# Autodesk Inventor assembly: タミヤダンパーフロント56,74.5
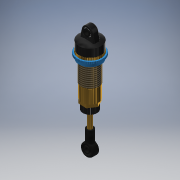
[picture p0: Inventor's stored thumbnail of the model, 180x180]
Saved by Autodesk Inventor 2020 (Build 240168000, 168)
## iProperties
Part Number: タミヤダンパーフロント56,74.5
Material: 一般
Document SubType Name: Assembly
Designer: 雪村
Mass: 29.9788 g
Surface Area: 59.981 cm^2
Volume: 5.28575 cm^3
Density: 5.67163 g/cm^3
Author: 雪村
## Documents named in this file (9)
- C:\Users\white\Documents\SRDC\SRDC\Inventor_2017\2018年機体\パーツ\タミヤダンパーフロント56,74.5.iam
- C:\Users\white\Documents\SRDC\SRDC\Inventor_2017\2018年機体\パーツ\タミヤダンパー1.ipt
- C:\Users\white\Documents\SRDC\SRDC\Inventor_2017\2018年機体\パーツ\タミヤダンパー2.ipt
- C:\Users\white\Documents\SRDC\SRDC\Inventor_2017\2018年機体\パーツ\タミヤダンパー3.ipt
- C:\Users\white\Documents\SRDC\SRDC\Inventor_2017\2018年機体\パーツ\タミヤダンパー4.ipt
- C:\Users\white\Documents\SRDC\SRDC\Inventor_2017\2018年機体\パーツ\タミヤダンパー6.ipt
- C:\Users\white\Documents\SRDC\SRDC\Inventor_2017\2018年機体\パーツ\タミヤダンパー5.ipt
- C:\Users\white\Documents\SRDC\SRDC\Inventor_2017\2018年機体\パーツ\タミヤダンパー7.ipt
- C:\Users\white\Documents\SRDC\SRDC\Inventor_2017\2018年機体\パーツ\タミヤダンパー8.ipt
## Components (9 placed, 8 different names)
1. タミヤダンパー1:1 — 挿入:1, 挿入:6
2. タミヤダンパー2:1 — 挿入:1, メイト:1, 挿入:4, 円柱状:1
3. タミヤダンパー3:1 — 挿入:3, 挿入:4
4. タミヤダンパー4:1 — メイト:1
5. タミヤダンパー6:1 — 挿入:3
6. タミヤダンパー5:1 — 円柱状:1, 挿入:7
7. タミヤダンパー7:1 — ボール:1, 挿入:7, メイト:2
8. タミヤダンパー8:1 — 挿入:6, フラッシュ:1
9. タミヤダンパー8:2 — ボール:1, フラッシュ:1, メイト:2
## Relationships (10: Insert 5, Mate 2, BallJoint 1, CylindricalJoint 1, Flush 1)
- 挿入:1 [Insert]: タミヤダンパー1:1 ↔ タミヤダンパー2:1
- メイト:1 [Mate]: タミヤダンパー2:1 ↔ タミヤダンパー4:1
- 挿入:3 [Insert]: タミヤダンパー3:1 ↔ タミヤダンパー6:1
- ボール:1 [BallJoint]: タミヤダンパー7:1 ↔ タミヤダンパー8:2
- 挿入:4 [Insert]: タミヤダンパー2:1 ↔ タミヤダンパー3:1
- 円柱状:1 [CylindricalJoint]: タミヤダンパー2:1 ↔ タミヤダンパー5:1
- 挿入:6 [Insert]: タミヤダンパー1:1 ↔ タミヤダンパー8:1
- 挿入:7 [Insert]: タミヤダンパー5:1 ↔ タミヤダンパー7:1
- フラッシュ:1 [Flush]: タミヤダンパー8:1 ↔ タミヤダンパー8:2
- メイト:2 [Mate]: タミヤダンパー7:1 ↔ タミヤダンパー8:2
## Named parameters: sa_0 = -220.283, sa_1 = -1.057e-09, sa_2 = 9997.57
note: some values were not read from the file. Shown as the stored number, unit unknown: "sa_0", "sa_1", "sa_2".
